# Autodesk Inventor assembly: Assembly_Rail_v2
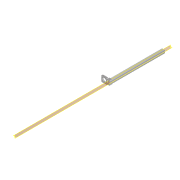
[picture p0: Inventor's stored thumbnail of the model, 180x180]
Saved by Autodesk Inventor 2022 (Build 260153000, 153)
## iProperties
Created: 2022-06-21
Part Number: Assembly_Rail_v2
Document SubType Name: Assembly
Designer: wanghaoran
Author: wanghaoran
## Documents named in this file (3)
- E:\GitHub\SIMMO\INVENTOR\Assembly_Rail_v2.iam
- E:\GitHub\SIMMO\INVENTOR\00_Aluminium_Extrusion_20x20.ipt
- E:\GitHub\SIMMO\INVENTOR\Rain_LensHolder.ipt
## Components (2 placed, 2 different names)
1. 00_Aluminium_Extrusion_20x20:1 — Flush:1
2. Rain_LensHolder:1 — Flush:1
## Relationships (1: Flush 1)
- Flush:1: 00_Aluminium_Extrusion_20x20:1 ↔ Rain_LensHolder:1
